# Autodesk Inventor assembly: touch screen model assembly
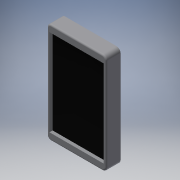
[picture p0: Inventor's stored thumbnail of the model, 180x180]
Saved by Autodesk Inventor 2018 (Build 220112000, 112)
## iProperties
Created: 2018-03-27
Part Number: touch screen model assembly
Document SubType Name: Assembly
Designer: Jacob
Title: C:\Users\moroz\Desktop\projects\SLS\корпус свой вариант\v3\электроника\raspberry pi display.stp
Author: moroz
Sending System: Autodesk Inventor 2017
Preprocessor: ST-DEVELOPER v16.5
## Documents named in this file (8)
- C:\Users\Jacob\Documents\IPRO 497\Alarm box parts\touch screen model assembly.iam
- C:\Users\Jacob\Downloads\raspberry-pi-display-7-1.snapshot.2\raspberry pi display.ipt
- C:\Users\Jacob\Downloads\raspberry-pi-display-7-1.snapshot.2\Raspberry Pi 3 .ipt
- C:\Users\Jacob\Downloads\raspberry-pi-display-7-1.snapshot.2\raspberry pi display module.ipt
- C:\Users\Jacob\Downloads\raspberry-pi-display-7-1.snapshot.2\стойка 12мм.ipt
- C:\Users\Jacob\Downloads\raspberry-pi-display-7-1.snapshot.2\cables.ipt
- C:\Users\Jacob\Downloads\raspberry-pi-display-7-1.snapshot.2\ISO 7045 - M2,5 x 3 - 4.8 - H - ISO.ipt
- C:\Users\Jacob\Documents\IPRO 497\Alarm box parts\Touch screen front box part.ipt
## Components (13 placed, 7 different names)
1. raspberry pi display:1 — Mate:2, Mate:3, Mate:4
2. Raspberry Pi 3 :1 — Mate:5
3. raspberry pi display module:1
4. стойка 12мм:1
5. стойка 12мм:2
6. стойка 12мм:3
7. стойка 12мм:4
8. cables:1
9. ISO 7045 H M2,5 x 3 - 4.8 - H:1
10. ISO 7045 H M2,5 x 3 - 4.8 - H:2
11. ISO 7045 H M2,5 x 3 - 4.8 - H:3
12. ISO 7045 H M2,5 x 3 - 4.8 - H:4 — Mate:5
13. Touch screen front box part:1 — Mate:2, Mate:3, Mate:4
## Relationships (4: Mate 4)
- Mate:2: raspberry pi display:1 ↔ Touch screen front box part:1
- Mate:3: raspberry pi display:1 ↔ Touch screen front box part:1
- Mate:4: raspberry pi display:1 ↔ Touch screen front box part:1
- Mate:5: Raspberry Pi 3 :1 ↔ ISO 7045 H M2,5 x 3 - 4.8 - H:4
